# Autodesk Inventor assembly: motor unit 2820
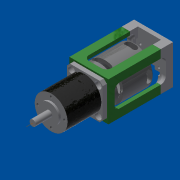
[picture p0: Inventor's stored thumbnail of the model, 180x180]
Saved by Autodesk Inventor 2018 (Build 220112000, 112)
## iProperties
Created: 2020-06-06
Part Number: motor unit 2820
Document SubType Name: Assembly
Designer: Bunny320
Author: Bunny320
## Documents named in this file (7)
- C:\Users\Bunny320\Desktop\sechs\4-CAD\motor unit 2820.iam
- C:\Users\Bunny320\Desktop\sechs\4-CAD\921-2820 house.ipt
- C:\Users\Bunny320\Desktop\sechs\4-CAD\standardParts\AS 2820 kv880\AS 2820 kv880.ipt
- C:\Users\Bunny320\Desktop\sechs\4-CAD\912-35-reducer.ipt
- C:\Users\Bunny320\Desktop\sechs\4-CAD\922-2820 magnet hold.ipt
- C:\Users\Bunny320\Desktop\sechs\4-CAD\923-2820 back.ipt
- C:\Users\Bunny320\Desktop\sechs\4-CAD\magnet-6x2.5.ipt
## Components (6 placed, 6 different names)
1. 921-2820 house:1 — Flush:1, Flush:2, Flush:3, Mate:1, Mate:2, Mate:3, Mate:4, Mate:5, Mate:6, Flush:4, Flush:5, Mate:12
2. AS 2820 kv880:1 — Mate:4, Mate:5, Mate:6, Mate:7, Mate:8, Mate:9
3. 912-35-reducer:1 — Mate:1, Mate:2, Mate:3
4. 922-2820 magnet hold:1 — Mate:7, Mate:8, Mate:9, Mate:13, Mate:14
5. 923-2820 back:1 — Flush:4, Flush:5, Mate:12
6. magnet-6x2.5:1 — Mate:13, Mate:14
## Relationships (17: Mate 12, Flush 5)
- Flush:1: 921-2820 house:1
- Flush:2: 921-2820 house:1
- Flush:3: 921-2820 house:1
- Mate:1: 921-2820 house:1 ↔ 912-35-reducer:1
- Mate:2: 921-2820 house:1 ↔ 912-35-reducer:1
- Mate:3: 921-2820 house:1 ↔ 912-35-reducer:1
- Mate:4: 921-2820 house:1 ↔ AS 2820 kv880:1
- Mate:5: 921-2820 house:1 ↔ AS 2820 kv880:1
- Mate:6: 921-2820 house:1 ↔ AS 2820 kv880:1
- Mate:7: AS 2820 kv880:1 ↔ 922-2820 magnet hold:1
- Mate:8: AS 2820 kv880:1 ↔ 922-2820 magnet hold:1
- Mate:9: AS 2820 kv880:1 ↔ 922-2820 magnet hold:1
- Flush:4: 921-2820 house:1 ↔ 923-2820 back:1
- Flush:5: 921-2820 house:1 ↔ 923-2820 back:1
- Mate:12: 921-2820 house:1 ↔ 923-2820 back:1
- Mate:13: 922-2820 magnet hold:1 ↔ magnet-6x2.5:1
- Mate:14: 922-2820 magnet hold:1 ↔ magnet-6x2.5:1
